# Autodesk Inventor assembly: inner rails 2
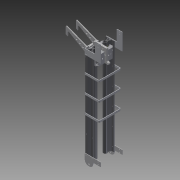
[picture p0: Inventor's stored thumbnail of the model, 180x180]
Saved by Autodesk Inventor 2013 (Build 170138000, 138)
## iProperties
Created: 2013-01-27
Part Number: inner rails 2
Document SubType Name: Assembly
Designer: Arpan
Mass: 6466.4 g
Surface Area: 8358.51 cm^2
Volume: 2006.35 cm^3
Density: 3.22296 g/cm^3
Author: Arpan
## Documents named in this file (7)
- C:\Users\Arpan\Documents\GitHub\frc2013CAD\Cimber actual\inner rails 2.iam
- C:\Users\Arpan\Documents\GitHub\frc2013CAD\Cimber actual\Shaft 26 inch.ipt
- C:\Users\Arpan\Documents\GitHub\frc2013CAD\Cimber actual\tie-together tier 1.ipt
- C:\Users\Arpan\Documents\GitHub\frc2013CAD\Cimber actual\hook block.iam
- C:\Users\Arpan\Documents\GitHub\frc2013CAD\Cimber actual\endstop 3.ipt
- C:\Users\Arpan\Documents\GitHub\frc2013CAD\Cimber actual\endstop 4.ipt
- C:\Users\Arpan\Documents\GitHub\frc2013CAD\Cimber actual\arm mout.ipt
## Components (10 placed, 6 different names)
1. Shaft 26 inch:1 — Angle:1, Flush:1, Mate:15, Mate:47, Mate:48, Mate:49, Mate:50, Mate:61, Mate:62, Mate:63, Mate:71, Mate:75, Mate:76, Mate:77
2. Shaft 26 inch:2 — Angle:1, Flush:1, Mate:46, Flush:2, Mate:51, Mate:52, Mate:53, Mate:59, Mate:60, Mate:67, Mate:68, Mate:69, Mate:70, Mate:72, Mate:73, Mate:74
3. tie-together tier 1:2 — Mate:15, Mate:68, Mate:71
4. tie-together tier 1:3 — Mate:59, Mate:60, Mate:69, Mate:70
5. hook block:1 [sub-assembly] — Mate:46, Mate:47, Flush:2
6. endstop 3:1 — Mate:51, Mate:52, Mate:53
7. endstop 4:1 — Mate:48, Mate:49, Mate:50
8. tie-together tier 1:4 — Mate:61, Mate:62, Mate:63, Mate:67
9. arm mout:1 — Mate:72, Mate:73, Mate:74
10. arm mout:2 — Mate:75, Mate:76, Mate:77
## Relationships (28: Mate 25, Flush 2, Angle 1)
- Angle:1 (180 deg): Shaft 26 inch:1 ↔ Shaft 26 inch:2
- Flush:1: Shaft 26 inch:1 ↔ Shaft 26 inch:2
- Mate:15: Shaft 26 inch:1 ↔ tie-together tier 1:2
- Mate:46: Shaft 26 inch:2 ↔ hook block:1
- Mate:47: Shaft 26 inch:1 ↔ hook block:1
- Flush:2 (558.8 mm): Shaft 26 inch:2 ↔ hook block:1
- Mate:48: Shaft 26 inch:1 ↔ endstop 4:1
- Mate:49: Shaft 26 inch:1 ↔ endstop 4:1
- Mate:50: Shaft 26 inch:1 ↔ endstop 4:1
- Mate:51: Shaft 26 inch:2 ↔ endstop 3:1
- Mate:52: Shaft 26 inch:2 ↔ endstop 3:1
- Mate:53: Shaft 26 inch:2 ↔ endstop 3:1
- Mate:59: Shaft 26 inch:2 ↔ tie-together tier 1:3
- Mate:60: Shaft 26 inch:2 ↔ tie-together tier 1:3
- Mate:61: Shaft 26 inch:1 ↔ tie-together tier 1:4
- Mate:62: Shaft 26 inch:1 ↔ tie-together tier 1:4
- Mate:63: Shaft 26 inch:1 ↔ tie-together tier 1:4
- Mate:67: Shaft 26 inch:2 ↔ tie-together tier 1:4
- Mate:68: Shaft 26 inch:2 ↔ tie-together tier 1:2
- Mate:69: Shaft 26 inch:2 ↔ tie-together tier 1:3
- Mate:70: Shaft 26 inch:2 ↔ tie-together tier 1:3
- Mate:71: Shaft 26 inch:1 ↔ tie-together tier 1:2
- Mate:72: Shaft 26 inch:2 ↔ arm mout:1
- Mate:73: Shaft 26 inch:2 ↔ arm mout:1
- Mate:74: Shaft 26 inch:2 ↔ arm mout:1
- Mate:75: Shaft 26 inch:1 ↔ arm mout:2
- Mate:76: Shaft 26 inch:1 ↔ arm mout:2
- Mate:77: Shaft 26 inch:1 ↔ arm mout:2
